# Autodesk Inventor assembly: Assembly1
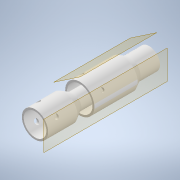
[picture p0: Inventor's stored thumbnail of the model, 180x180]
Saved by Autodesk Inventor 2021 (Build 250183000, 183)
## iProperties
Created: 2023-07-02
Part Number: Assembly1
Document SubType Name: Assembly
Designer: harsh
Author: harsh
## Documents named in this file (3)
- C:\Users\harsh\Documents\Course 7th sem\internship\simulation\CAD\Assembly1.iam
- C:\Users\harsh\Documents\Course 7th sem\internship\simulation\CAD\fuel.ipt
- C:\Users\harsh\Documents\Course 7th sem\internship\simulation\CAD\oxidizer.ipt
## Components (2 placed, 2 different names)
1. fuel:1 — Mate:1, Flush:1
2. oxidizer:1 — Mate:1, Flush:1
## Relationships (2: Mate 1, Flush 1)
- Mate:1: fuel:1 ↔ oxidizer:1
- Flush:1 (1 mm): fuel:1 ↔ oxidizer:1
